# Autodesk Inventor assembly: ROBOT_1_4
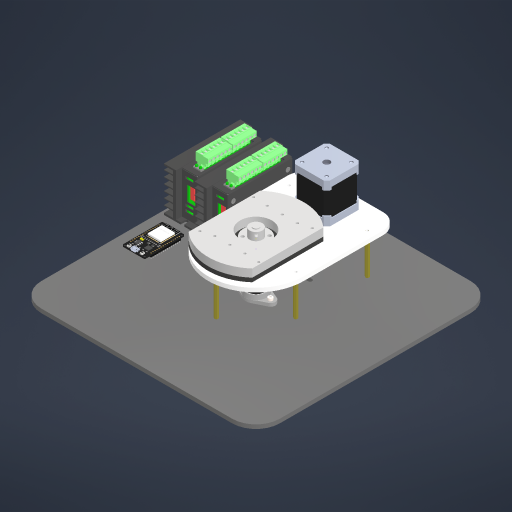
[picture p0: Inventor's stored thumbnail of the model, 512x512]
Saved by Autodesk Inventor 2023 (Build 270158000, 158)
## iProperties
Created: 2023-09-06
Part Number: ROBOT_1_4
Document SubType Name: Assembly
Designer: philo
Sending System: Autodesk Inventor 2023
Preprocessor: ST-DEVELOPER v19
Title: C:\Users\philo\OneDrive\Desktop\HK1-2024\TT ROBOT\3DVer2\ROBOT_1_2.stp
Author: philo
## Documents named in this file (20)
- C:\Users\philo\OneDrive\Desktop\HK1-2024\TT ROBOT\02_3D_design_new\ROBOT_1_4.iam
- C:\Users\philo\OneDrive\Desktop\HK1-2024\TT ROBOT\02_3D_design_new\DeRobot.ipt
- C:\Users\philo\OneDrive\Desktop\HK1-2024\TT ROBOT\02_3D_design_new\Detron.ipt
- C:\Users\philo\OneDrive\Desktop\HK1-2024\TT ROBOT\02_3D_design_new\goidoObi.ipt
- C:\Users\philo\OneDrive\Desktop\HK1-2024\TT ROBOT\02_3D_design_new\truday.ipt
- C:\Users\philo\OneDrive\Desktop\HK1-2024\TT ROBOT\02_3D_design_new\gt2_60teeth.iam
- C:\Users\philo\OneDrive\Desktop\HK1-2024\TT ROBOT\02_3D_design_new\STEP MOTOR NEMA 17.ipt
- C:\Users\philo\OneDrive\Desktop\HK1-2024\TT ROBOT\02_3D_design_new\GT2 Pulley 20 Tooth (ID6mm).ipt
- C:\Users\philo\OneDrive\Desktop\HK1-2024\TT ROBOT\02_3D_design_new\M3 x 5mm.ipt
- C:\Users\philo\OneDrive\Desktop\HK1-2024\TT ROBOT\02_3D_design_new\Diaquay.ipt
- C:\Users\philo\OneDrive\Desktop\HK1-2024\TT ROBOT\02_3D_design_new\Tb6600.ipt
- C:\Users\philo\OneDrive\Desktop\HK1-2024\TT ROBOT\02_3D_design_new\ESP-WROOM32.iam
- C:\Users\philo\OneDrive\Desktop\HK1-2024\TT ROBOT\02_3D_design_new\codinhtruc.ipt
- C:\Users\philo\OneDrive\Desktop\HK1-2024\TT ROBOT\02_3D_design_new\daydai.ipt
- C:\Users\philo\OneDrive\Desktop\HK1-2024\TT ROBOT\02_3D_design_new\gt2smooth.ipt
- C:\Users\philo\OneDrive\Desktop\HK1-2024\TT ROBOT\02_3D_design_new\trudong5mm.ipt
- C:\Users\philo\OneDrive\Desktop\HK1-2024\TT ROBOT\02_3D_design_new\trucdogt2.ipt
- C:\Users\philo\OneDrive\Desktop\HK1-2024\TT ROBOT\02_3D_design_new\HALL.ipt
- C:\Users\philo\OneDrive\Desktop\HK1-2024\TT ROBOT\02_3D_design_new\namcham.ipt
- C:\Users\philo\OneDrive\Desktop\HK1-2024\TT ROBOT\02_3D_design\Part1.ipt
## Components (28 placed, 19 different names)
1. DeRobot:1 — Mate:81, Mate:82, Mate:83, Mate:84, Mate:85, Mate:86, Mate:87, Mate:90, Mate:91, Mate:92, Mate:95, Flush:16, Mate:174, Mate:175
2. Detron:1 — Mate:33, Mate:81, Mate:94, Mate:95, Mate:96, Mate:97, Angle:11
3. goidoObi:1 — Mate:93, Mate:94
4. goidoObi:2 — Mate:89, Mate:92
5. truday:1 — Mate:32, Mate:87, Mate:88, Mate:93, Flush:16
6. gt2_60teeth:1 [sub-assembly] — Mate:88, Mate:89
7. STEP MOTOR NEMA 17:1 — Mate:96, Mate:97, Angle:11, Mate:98
8. GT2 Pulley 20 Tooth (ID6mm):1 — Mate:98
9. M3 x 5mm:1
10. M3 x 5mm:6
11. M3 x 5mm:7 — Mate:90
12. M3 x 5mm:8 — Mate:91
13. Tb6600:1 — Mate:174
14. Tb6600:2 — Mate:175
15. ESP-WROOM32:1 [sub-assembly]
16. daydai:1
17. gt2smooth:1 — Mate:99
18. trudong5mm:4 — Mate:84
19. trudong5mm:5 — Mate:82
20. trudong5mm:6 — Mate:85
21. trudong5mm:8 — Mate:86
22. trudong5mm:9 — Mate:83
23. trucdogt2:1 — Mate:99
24. HALL:1
25. Diaquay:1 — Mate:1, Mate:2, Mate:32, Mate:33, Mate:34, Flush:3, Mate:116, Mate:117, Flush:18, Flush:19
26. codinhtruc:2 — Mate:1, Mate:2, Mate:34
27. namcham:1 — Flush:3, Mate:116, Mate:117
28. Part1:1 — Flush:18, Flush:19
## Relationships (33: Mate 28, Flush 4, Angle 1)
- Mate:1: Diaquay:1 ↔ codinhtruc:2
- Mate:2: Diaquay:1 ↔ codinhtruc:2
- Mate:32: truday:1 ↔ Diaquay:1
- Mate:33 (6 mm): Detron:1 ↔ Diaquay:1
- Mate:34: Diaquay:1 ↔ codinhtruc:2
- Flush:3: Diaquay:1 ↔ namcham:1
- Mate:81 (45 mm): DeRobot:1 ↔ Detron:1
- Mate:82: DeRobot:1 ↔ trudong5mm:5
- Mate:83: DeRobot:1 ↔ trudong5mm:9
- Mate:84: DeRobot:1 ↔ trudong5mm:4
- Mate:85: DeRobot:1 ↔ trudong5mm:6
- Mate:86: DeRobot:1 ↔ trudong5mm:8
- Mate:87: DeRobot:1 ↔ truday:1
- Mate:88: truday:1 ↔ gt2_60teeth:1
- Mate:89: goidoObi:2 ↔ gt2_60teeth:1
- Mate:90: DeRobot:1 ↔ M3 x 5mm:7
- Mate:91: DeRobot:1 ↔ M3 x 5mm:8
- Mate:92: DeRobot:1 ↔ goidoObi:2
- Mate:93: goidoObi:1 ↔ truday:1
- Mate:94: Detron:1 ↔ goidoObi:1
- Mate:95: DeRobot:1 ↔ Detron:1
- Mate:96: Detron:1 ↔ STEP MOTOR NEMA 17:1
- Mate:97: Detron:1 ↔ STEP MOTOR NEMA 17:1
- Angle:11 (0 deg): Detron:1 ↔ STEP MOTOR NEMA 17:1
- Mate:98: STEP MOTOR NEMA 17:1 ↔ GT2 Pulley 20 Tooth (ID6mm):1
- Mate:99: gt2smooth:1 ↔ trucdogt2:1
- Mate:116: Diaquay:1 ↔ namcham:1
- Mate:117 (60 mm): Diaquay:1 ↔ namcham:1
- Flush:16: DeRobot:1 ↔ truday:1
- Flush:18: Diaquay:1 ↔ Part1:1
- Flush:19: Diaquay:1 ↔ Part1:1
- Mate:174: DeRobot:1 ↔ Tb6600:1
- Mate:175: DeRobot:1 ↔ Tb6600:2
